# Autodesk Inventor assembly: waterjet assembly version
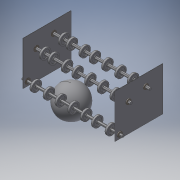
[picture p0: Inventor's stored thumbnail of the model, 180x180]
Saved by Autodesk Inventor 2018 (Build 220112000, 112)
## iProperties
Created: 2020-01-24
Part Number: waterjet assembly version
Document SubType Name: Assembly
Designer: s-2513225
Author: s-2513225
## Documents named in this file (6)
- \\studenthome\students\S-2513225\GitHub\2020CAD\Over bumper intake\Assembly\waterjet assembly version.iam
- \\studenthome\students\S-2513225\GitHub\2020CAD\Over bumper intake\Parts\waterjet wall.ipt
- \\studenthome\students\S-2513225\GitHub\2020CAD\Over bumper intake\Parts\0_500_Hex_ID_x_1_125_OD_x_0_313_WD_Flanged_Bearing_v2_217-3875.ipt
- \\studenthome\students\S-2513225\GitHub\2020CAD\Over bumper intake\Parts\hex shaft 1.ipt
- \\studenthome\students\S-2513225\GitHub\2020CAD\Over bumper intake\Parts\ball mock up.ipt
- \\studenthome\students\S-2513225\GitHub\2020CAD\Over bumper intake\Parts\banebots 400 - 2 3-8 replacement.ipt
## Components (33 placed, 5 different names)
1. waterjet wall:1 — Mate:1, Mate:2, Mate:3, Mate:4, Mate:5, Mate:6, Mate:7, Mate:8, Mate:9, Mate:26
2. waterjet wall:2 — Mate:16, Mate:17, Mate:18, Mate:19, Mate:20, Mate:21, Mate:22, Mate:26
3. 0_500_Hex_ID_x_1_125_OD_x_0_313_WD_Flanged_Bearing_v2_217-3875:1 — Mate:5, Mate:7, Mate:10, Mate:15
4. 0_500_Hex_ID_x_1_125_OD_x_0_313_WD_Flanged_Bearing_v2_217-3875:2 — Mate:6, Mate:9, Mate:12, Mate:14
5. 0_500_Hex_ID_x_1_125_OD_x_0_313_WD_Flanged_Bearing_v2_217-3875:3 — Mate:4, Mate:8, Mate:11, Mate:13
6. 0_500_Hex_ID_x_1_125_OD_x_0_313_WD_Flanged_Bearing_v2_217-3875:4 — Mate:19, Mate:21, Mate:24
7. 0_500_Hex_ID_x_1_125_OD_x_0_313_WD_Flanged_Bearing_v2_217-3875:5 — Mate:18, Mate:20, Mate:23, Mate:25
8. 0_500_Hex_ID_x_1_125_OD_x_0_313_WD_Flanged_Bearing_v2_217-3875:6 — Mate:17, Mate:22
9. hex shaft 1:1 — Mate:12, Mate:14, Mate:23, Mate:25, Mate:35, Mate:37, Mate:53, Mate:54, Mate:59, Mate:60, Mate:68, Mate:72, Mate:73, Mate:74, Mate:75, Mate:76, Mate:77, Mate:78
10. hex shaft 1:2 — Mate:10, Mate:15, Mate:27, Mate:28, Mate:29, Mate:30, Mate:39, Mate:42, Mate:43, Mate:44, Mate:45, Mate:46, Mate:61, Mate:62, Mate:63, Mate:64
11. hex shaft 1:3 — Mate:11, Mate:13, Mate:24, Mate:31, Mate:32, Mate:33, Mate:34, Mate:40, Mate:47, Mate:48, Mate:49, Mate:50, Mate:51, Mate:65, Mate:66, Mate:69, Mate:70
12. ball mock up:1
13. banebots 400 - 2 3-8 replacement:1 — Mate:27, Mate:42
14. banebots 400 - 2 3-8 replacement:2 — Mate:30, Mate:43
15. banebots 400 - 2 3-8 replacement:3 — Mate:31, Mate:50
16. banebots 400 - 2 3-8 replacement:4 — Mate:29, Mate:44
17. banebots 400 - 2 3-8 replacement:5 — Mate:40, Mate:51
18. banebots 400 - 2 3-8 replacement:6 — Mate:28, Mate:46
19. banebots 400 - 2 3-8 replacement:7 — Mate:34, Mate:47
20. banebots 400 - 2 3-8 replacement:8 — Mate:32, Mate:48
21. banebots 400 - 2 3-8 replacement:9 — Mate:39, Mate:45
22. banebots 400 - 2 3-8 replacement:10 — Mate:73, Mate:78
23. banebots 400 - 2 3-8 replacement:11 — Mate:37, Mate:53
24. banebots 400 - 2 3-8 replacement:12 — Mate:75, Mate:76
25. banebots 400 - 2 3-8 replacement:13 — Mate:35, Mate:54
26. banebots 400 - 2 3-8 replacement:14 — Mate:33, Mate:49
27. banebots 400 - 2 3-8 replacement:15 — Mate:59, Mate:60
28. banebots 400 - 2 3-8 replacement:16 — Mate:61, Mate:63
29. banebots 400 - 2 3-8 replacement:17 — Mate:62, Mate:64
30. banebots 400 - 2 3-8 replacement:18 — Mate:66, Mate:70
31. banebots 400 - 2 3-8 replacement:19 — Mate:65, Mate:69
32. banebots 400 - 2 3-8 replacement:20 — Mate:74, Mate:77
33. banebots 400 - 2 3-8 replacement:21 — Mate:68, Mate:72
## Relationships (68: Mate 68)
- Mate:1: waterjet wall:1
- Mate:2: waterjet wall:1
- Mate:3: waterjet wall:1
- Mate:4: waterjet wall:1 ↔ 0_500_Hex_ID_x_1_125_OD_x_0_313_WD_Flanged_Bearing_v2_217-3875:3
- Mate:5: waterjet wall:1 ↔ 0_500_Hex_ID_x_1_125_OD_x_0_313_WD_Flanged_Bearing_v2_217-3875:1
- Mate:6: waterjet wall:1 ↔ 0_500_Hex_ID_x_1_125_OD_x_0_313_WD_Flanged_Bearing_v2_217-3875:2
- Mate:7: waterjet wall:1 ↔ 0_500_Hex_ID_x_1_125_OD_x_0_313_WD_Flanged_Bearing_v2_217-3875:1
- Mate:8: waterjet wall:1 ↔ 0_500_Hex_ID_x_1_125_OD_x_0_313_WD_Flanged_Bearing_v2_217-3875:3
- Mate:9: waterjet wall:1 ↔ 0_500_Hex_ID_x_1_125_OD_x_0_313_WD_Flanged_Bearing_v2_217-3875:2
- Mate:10: 0_500_Hex_ID_x_1_125_OD_x_0_313_WD_Flanged_Bearing_v2_217-3875:1 ↔ hex shaft 1:2
- Mate:11: 0_500_Hex_ID_x_1_125_OD_x_0_313_WD_Flanged_Bearing_v2_217-3875:3 ↔ hex shaft 1:3
- Mate:12: 0_500_Hex_ID_x_1_125_OD_x_0_313_WD_Flanged_Bearing_v2_217-3875:2 ↔ hex shaft 1:1
- Mate:13: 0_500_Hex_ID_x_1_125_OD_x_0_313_WD_Flanged_Bearing_v2_217-3875:3 ↔ hex shaft 1:3
- Mate:14: 0_500_Hex_ID_x_1_125_OD_x_0_313_WD_Flanged_Bearing_v2_217-3875:2 ↔ hex shaft 1:1
- Mate:15: 0_500_Hex_ID_x_1_125_OD_x_0_313_WD_Flanged_Bearing_v2_217-3875:1 ↔ hex shaft 1:2
- Mate:16: waterjet wall:2
- Mate:17: waterjet wall:2 ↔ 0_500_Hex_ID_x_1_125_OD_x_0_313_WD_Flanged_Bearing_v2_217-3875:6
- Mate:18: waterjet wall:2 ↔ 0_500_Hex_ID_x_1_125_OD_x_0_313_WD_Flanged_Bearing_v2_217-3875:5
- Mate:19: waterjet wall:2 ↔ 0_500_Hex_ID_x_1_125_OD_x_0_313_WD_Flanged_Bearing_v2_217-3875:4
- Mate:20: waterjet wall:2 ↔ 0_500_Hex_ID_x_1_125_OD_x_0_313_WD_Flanged_Bearing_v2_217-3875:5
- Mate:21: waterjet wall:2 ↔ 0_500_Hex_ID_x_1_125_OD_x_0_313_WD_Flanged_Bearing_v2_217-3875:4
- Mate:22: waterjet wall:2 ↔ 0_500_Hex_ID_x_1_125_OD_x_0_313_WD_Flanged_Bearing_v2_217-3875:6
- Mate:23: 0_500_Hex_ID_x_1_125_OD_x_0_313_WD_Flanged_Bearing_v2_217-3875:5 ↔ hex shaft 1:1
- Mate:24: 0_500_Hex_ID_x_1_125_OD_x_0_313_WD_Flanged_Bearing_v2_217-3875:4 ↔ hex shaft 1:3
- Mate:25: 0_500_Hex_ID_x_1_125_OD_x_0_313_WD_Flanged_Bearing_v2_217-3875:5 ↔ hex shaft 1:1
- Mate:26 (533.4 mm): waterjet wall:1 ↔ waterjet wall:2
- Mate:27: hex shaft 1:2 ↔ banebots 400 - 2 3-8 replacement:1
- Mate:28: hex shaft 1:2 ↔ banebots 400 - 2 3-8 replacement:6
- Mate:29: hex shaft 1:2 ↔ banebots 400 - 2 3-8 replacement:4
- Mate:30: hex shaft 1:2 ↔ banebots 400 - 2 3-8 replacement:2
- Mate:31: hex shaft 1:3 ↔ banebots 400 - 2 3-8 replacement:3
- Mate:32: hex shaft 1:3 ↔ banebots 400 - 2 3-8 replacement:8
- Mate:33: hex shaft 1:3 ↔ banebots 400 - 2 3-8 replacement:14
- Mate:34: hex shaft 1:3 ↔ banebots 400 - 2 3-8 replacement:7
- Mate:35: hex shaft 1:1 ↔ banebots 400 - 2 3-8 replacement:13
- Mate:37: hex shaft 1:1 ↔ banebots 400 - 2 3-8 replacement:11
- Mate:39: hex shaft 1:2 ↔ banebots 400 - 2 3-8 replacement:9
- Mate:40: hex shaft 1:3 ↔ banebots 400 - 2 3-8 replacement:5
- Mate:42: hex shaft 1:2 ↔ banebots 400 - 2 3-8 replacement:1
- Mate:43: hex shaft 1:2 ↔ banebots 400 - 2 3-8 replacement:2
- Mate:44: hex shaft 1:2 ↔ banebots 400 - 2 3-8 replacement:4
- Mate:45: hex shaft 1:2 ↔ banebots 400 - 2 3-8 replacement:9
- Mate:46: hex shaft 1:2 ↔ banebots 400 - 2 3-8 replacement:6
- Mate:47: hex shaft 1:3 ↔ banebots 400 - 2 3-8 replacement:7
- Mate:48: hex shaft 1:3 ↔ banebots 400 - 2 3-8 replacement:8
- Mate:49: hex shaft 1:3 ↔ banebots 400 - 2 3-8 replacement:14
- Mate:50: hex shaft 1:3 ↔ banebots 400 - 2 3-8 replacement:3
- Mate:51: hex shaft 1:3 ↔ banebots 400 - 2 3-8 replacement:5
- Mate:53: hex shaft 1:1 ↔ banebots 400 - 2 3-8 replacement:11
- Mate:54: hex shaft 1:1 ↔ banebots 400 - 2 3-8 replacement:13
- Mate:59: hex shaft 1:1 ↔ banebots 400 - 2 3-8 replacement:15
- Mate:60: hex shaft 1:1 ↔ banebots 400 - 2 3-8 replacement:15
- Mate:61: hex shaft 1:2 ↔ banebots 400 - 2 3-8 replacement:16
- Mate:62: hex shaft 1:2 ↔ banebots 400 - 2 3-8 replacement:17
- Mate:63: hex shaft 1:2 ↔ banebots 400 - 2 3-8 replacement:16
- Mate:64: hex shaft 1:2 ↔ banebots 400 - 2 3-8 replacement:17
- Mate:65: hex shaft 1:3 ↔ banebots 400 - 2 3-8 replacement:19
- Mate:66: hex shaft 1:3 ↔ banebots 400 - 2 3-8 replacement:18
- Mate:68: hex shaft 1:1 ↔ banebots 400 - 2 3-8 replacement:21
- Mate:69: hex shaft 1:3 ↔ banebots 400 - 2 3-8 replacement:19
- Mate:70: hex shaft 1:3 ↔ banebots 400 - 2 3-8 replacement:18
- Mate:72: hex shaft 1:1 ↔ banebots 400 - 2 3-8 replacement:21
- Mate:73: hex shaft 1:1 ↔ banebots 400 - 2 3-8 replacement:10
- Mate:74: hex shaft 1:1 ↔ banebots 400 - 2 3-8 replacement:20
- Mate:75: hex shaft 1:1 ↔ banebots 400 - 2 3-8 replacement:12
- Mate:76: hex shaft 1:1 ↔ banebots 400 - 2 3-8 replacement:12
- Mate:77: hex shaft 1:1 ↔ banebots 400 - 2 3-8 replacement:20
- Mate:78: hex shaft 1:1 ↔ banebots 400 - 2 3-8 replacement:10
